# Autodesk Inventor assembly: Assembly Macaco
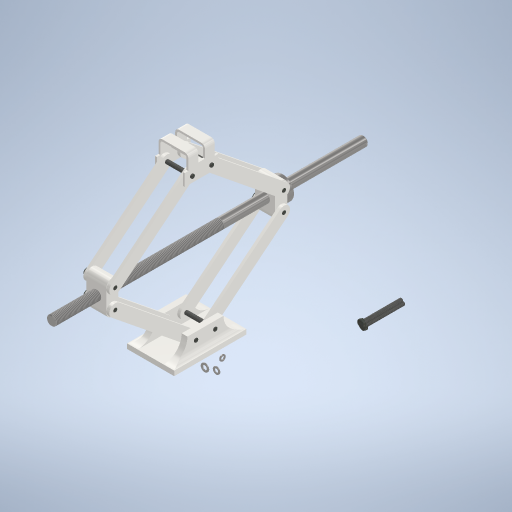
[picture p0: Inventor's stored thumbnail of the model, 512x512]
Saved by Autodesk Inventor 2024 (Build 280153000, 153)
## iProperties
Created: 2024-06-01
Part Number: Assembly Macaco
Document SubType Name: Assembly
Designer: Pedro
d10: 0,000 mm
w_Braço: 12,000 mm
Author: Pedro
## Documents named in this file (20)
- C:\Users\Pedro\Desktop\Autodesk Inbentor\Projeto\Assembly Macaco.iam
- C:\Users\Pedro\Desktop\Autodesk Inbentor\Projeto\Base Macaco.ipt
- C:\Users\Pedro\Desktop\Autodesk Inbentor\Projeto\Braço Macaco.ipt
- C:\Users\Pedro\Desktop\Autodesk Inbentor\Projeto\Junção Fuso.ipt
- C:\Users\Pedro\Desktop\Autodesk Inbentor\Projeto\Encaixe Macaco.ipt
- C:\Users\Pedro\Documents\Inventor\Content Center Files\R2024\en-US\DIN 615\DIN 615 - E 20 - 20 x 47 x 12.ipt
- C:\Users\Pedro\Desktop\Autodesk Inbentor\Projeto\DIN 427 - M20 x 650.ipt
- C:\Users\Pedro\Documents\Inventor\Content Center Files\R2024\en-US\ISO 4018\ISO 4018 - M8 x 80.ipt
- C:\Users\Pedro\Desktop\Autodesk Inbentor\Projeto\ISO 4018 - M8 x 80.ipt
- C:\Users\Pedro\Documents\Inventor\Content Center Files\R2024\en-US\ISO 4018\ISO 4018 - M8 x 55.ipt
- C:\Users\Pedro\Documents\Inventor\Content Center Files\R2024\en-US\ISO 7089\ISO 7089 - 6 - 140 HV(1).ipt
- C:\Users\Pedro\Documents\Inventor\Content Center Files\R2024\en-US\DIN 126\DIN 126 - 9.ipt
- C:\Users\Pedro\Documents\Inventor\Content Center Files\R2024\en-US\DIN 126\DIN 126 - 7,6.ipt
- C:\Users\Pedro\Documents\Inventor\Content Center Files\R2024\en-US\ISO 4018\ISO 4018 - M8 x 65.ipt
- C:\Users\Pedro\Desktop\Autodesk Inbentor\Projeto\Assembly Macaco\AIP\FEA\epzg9a0f4.fins
- C:\Users\Pedro\Desktop\Autodesk Inbentor\Projeto\Assembly Macaco\AIP\FEA\epzg9a0g0.fsat
- C:\Users\Pedro\Desktop\Autodesk Inbentor\Projeto\Assembly Macaco\AIP\FEA\epzg9a0g0.ftes
- C:\Users\Pedro\Desktop\Autodesk Inbentor\Projeto\Assembly Macaco\AIP\FEA\epzg9a0g0.fwiz
- C:\Users\Pedro\Desktop\Autodesk Inbentor\Projeto\Assembly Macaco\AIP\FEA\epzg9a0m8.fmsh
- C:\Users\Pedro\Desktop\Autodesk Inbentor\Projeto\Assembly Macaco\AIP\FEA\epzg9a0m9.fres
## Components (27 placed, 13 different names)
1. Base Macaco:1 — Insert:5, Insert:6, Insert:7, Insert:33, Angle:2, Angle:3, Mate:14, Insert:51, Insert:52
2. Braço Macaco:2 — Insert:5, Insert:9
3. Braço Macaco:3 — Insert:6, Insert:10, Insert:55
4. Braço Macaco:4 — Insert:7, Insert:53, Insert:59
5. Junção Fuso:1 — Insert:9, Insert:14, Insert:15, Angle:1, Mate:2, Mate:8, Insert:59
6. Junção Fuso:2 — Insert:10, Angle:1, Angle:2, Mate:2, Mate:4, Mate:6, Mate:7, Insert:41, Insert:42
7. Braço Macaco:5 — Insert:31, Mate:7
8. Braço Macaco:6 — Insert:14, Insert:32
9. Braço Macaco:7 — Mate:6, Insert:46, Insert:56
10. Braço Macaco:8 — Insert:15, Insert:50, Insert:54
11. Encaixe Macaco:1 — Insert:31, Insert:32, Angle:3, Insert:46, Insert:50, Mate:14, Insert:57, Insert:58
12. Braço Macaco:9 — Insert:33, Mate:4
13. DIN 615 E 20 - 20 x 47 x 12:1 — Insert:42
14. DIN 427 - M20 x 650:1 — Insert:41, Mate:8
15. ISO 4018 - M8 x 80:3
16. ISO 4018 - M8 x 80:4
17. ISO 4018 M8 x 80:1 — Insert:51
18. ISO 7089 6:1
19. DIN 126 9:1
20. DIN 126 7,6:1
21. ISO 4018 M8 x 80:2 — Insert:52
22. ISO 4018 M8 x 55:1 — Insert:53
23. ISO 4018 M8 x 55:2 — Insert:54
24. ISO 4018 M8 x 55:5 — Insert:55
25. ISO 4018 M8 x 55:6 — Insert:56
26. ISO 4018 M8 x 65:1 — Insert:57
27. ISO 4018 M8 x 65:2 — Insert:58
## Relationships (32: Insert 23, Mate 6, Angle 3)
- Insert:5: Base Macaco:1 ↔ Braço Macaco:2
- Insert:6: Base Macaco:1 ↔ Braço Macaco:3
- Insert:7: Base Macaco:1 ↔ Braço Macaco:4
- Insert:9: Braço Macaco:2 ↔ Junção Fuso:1
- Insert:10: Braço Macaco:3 ↔ Junção Fuso:2
- Insert:14: Junção Fuso:1 ↔ Braço Macaco:6
- Insert:15: Junção Fuso:1 ↔ Braço Macaco:8
- Insert:31: Braço Macaco:5 ↔ Encaixe Macaco:1
- Insert:32: Braço Macaco:6 ↔ Encaixe Macaco:1
- Insert:33: Base Macaco:1 ↔ Braço Macaco:9
- Angle:1 (180 deg): Junção Fuso:1 ↔ Junção Fuso:2
- Angle:2 (0 deg): Base Macaco:1 ↔ Junção Fuso:2
- Mate:2 (252.272 mm): Junção Fuso:1 ↔ Junção Fuso:2
- Mate:4: Junção Fuso:2 ↔ Braço Macaco:9
- Mate:6: Junção Fuso:2 ↔ Braço Macaco:7
- Mate:7: Junção Fuso:2 ↔ Braço Macaco:5
- Insert:41 (-175 mm): Junção Fuso:2 ↔ DIN 427 - M20 x 650:1
- Mate:8: Junção Fuso:1 ↔ DIN 427 - M20 x 650:1
- Insert:42: Junção Fuso:2 ↔ DIN 615 E 20 - 20 x 47 x 12:1
- Angle:3 (0 deg): Base Macaco:1 ↔ Encaixe Macaco:1
- Insert:46: Braço Macaco:7 ↔ Encaixe Macaco:1
- Insert:50: Braço Macaco:8 ↔ Encaixe Macaco:1
- Mate:14 (262.575 mm): Base Macaco:1 ↔ Encaixe Macaco:1
- Insert:51: Base Macaco:1 ↔ ISO 4018 M8 x 80:1
- Insert:52: Base Macaco:1 ↔ ISO 4018 M8 x 80:2
- Insert:53: Braço Macaco:4 ↔ ISO 4018 M8 x 55:1
- Insert:54: Braço Macaco:8 ↔ ISO 4018 M8 x 55:2
- Insert:55: Braço Macaco:3 ↔ ISO 4018 M8 x 55:5
- Insert:56: Braço Macaco:7 ↔ ISO 4018 M8 x 55:6
- Insert:57: Encaixe Macaco:1 ↔ ISO 4018 M8 x 65:1
- Insert:58: Encaixe Macaco:1 ↔ ISO 4018 M8 x 65:2
- Insert:59: Braço Macaco:4 ↔ Junção Fuso:1
## Named parameters: sa_0 = 1962
note: some values were not read from the file. Shown as the stored number, unit unknown: "sa_0".
